# Autodesk Inventor assembly: VL53L0X_assembly_1
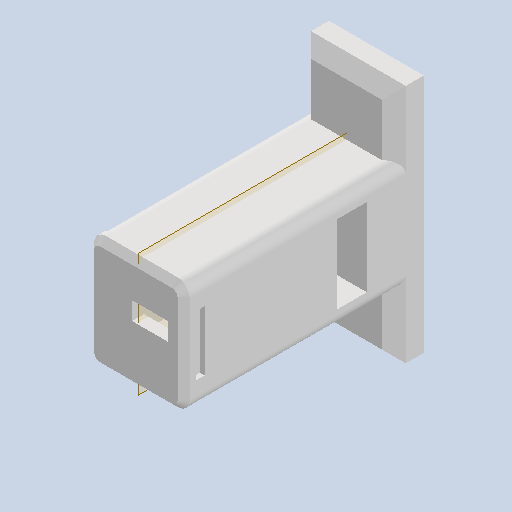
[picture p0: Inventor's stored thumbnail of the model, 512x512]
Saved by Autodesk Inventor 2025.3 (Build 293356000, 356)
## iProperties
Created: 2025-11-14
Part Number: VL53L0X_assembly_1
Document SubType Name: Assembly
Designer: woyao
Author: woyao
## Documents named in this file (3)
- D:\Sabi\gogogo\KIT\Hiwi\WBK_Mikrocontroller\Lasersensor+MQTT\Sensor\sensor_demo_1\VL53L0X_assembly_1.iam
- D:\Sabi\gogogo\KIT\Hiwi\WBK_Mikrocontroller\Lasersensor+MQTT\Sensor\sensor_demo_1\VL53L0X_case.ipt
- D:\Sabi\gogogo\KIT\Hiwi\WBK_Mikrocontroller\Lasersensor+MQTT\Sensor\sensor_demo_1\VL53L0X_cover.ipt
## Components (2 placed, 2 different names)
1. VL53L0X_case:1 — Mate:2, Mate:3, Mate:4, Mate:5
2. VL53L0X_cover:1 — Mate:2, Mate:3, Mate:4
## Relationships (4: Mate 4)
- Mate:2: VL53L0X_case:1 ↔ VL53L0X_cover:1
- Mate:3: VL53L0X_case:1 ↔ VL53L0X_cover:1
- Mate:4: VL53L0X_case:1 ↔ VL53L0X_cover:1
- Mate:5: VL53L0X_case:1
